# Autodesk Inventor assembly: Helmet_paneletchtool_200114_v01_nosurftol_origin
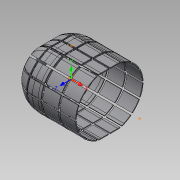
[picture p0: Inventor's stored thumbnail of the model, 180x180]
Saved by Autodesk Inventor 2018 (Build 220112000, 112)
## iProperties
Created: 2020-01-20
Part Number: Helmet_paneletchtool_200114_v01_nosurftol_origin
Document SubType Name: Assembly
Designer: pm589
Author: pm589
## Documents named in this file (2)
- C:\Users\pm589\Dropbox (MIT)\MRI\HelmetMagnet\CAD\RFCoil\Helmet_paneletchtool_200114_v01_nosurftol_origin.iam
- C:\Users\pm589\Dropbox (MIT)\MRI\HelmetMagnet\CAD\RFCoil\Helmet_paneletchtool_200114_v01_nosurftol_UCS.ipt
## Components (1 placed, 1 different names)
1. Helmet_paneletchtool_200114_v01_nosurftol_UCS:1 — Flush:1, Flush:2, Flush:3
## Relationships (3: Flush 3)
- Flush:1: Helmet_paneletchtool_200114_v01_nosurftol_UCS:1
- Flush:2: Helmet_paneletchtool_200114_v01_nosurftol_UCS:1
- Flush:3: Helmet_paneletchtool_200114_v01_nosurftol_UCS:1
